# Autodesk Inventor assembly: chassis weldment bottom
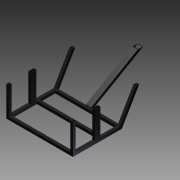
[picture p0: Inventor's stored thumbnail of the model, 180x180]
Saved by Autodesk Inventor 2012 (Build 160160000, 160)
## iProperties
Created: 2011-09-30
Part Number: chassis weldment bottom
Document SubType Name: Weldment
Designer: Antonella
Weld Material: Welded Aluminum-6061
Author: Antonella
## Documents named in this file (9)
- C:\Users\Antonella\Documents\GCC Robotics 2012 - Mechanical\Robot 2.0\Chassis\chassis weldment bottom.iam
- C:\Users\Antonella\Documents\GCC Robotics 2012 - Mechanical\Robot 2.0\Chassis\bottom frame member side.ipt
- C:\Users\Antonella\Documents\GCC Robotics 2012 - Mechanical\Robot 2.0\Chassis\bottom frame member crossbrace.ipt
- C:\Users\Antonella\Documents\GCC Robotics 2012 - Mechanical\Robot 2.0\Chassis\bottom frame member side_MIR.ipt
- C:\Users\Antonella\Documents\GCC Robotics 2012 - Mechanical\Robot 2.0\Chassis\bottom frame member angle.ipt
- C:\Users\Antonella\Documents\GCC Robotics 2012 - Mechanical\Robot 2.0\Chassis\bottom frame member back upright.ipt
- C:\Users\Antonella\Documents\GCC Robotics 2012 - Mechanical\Robot 2.0\Chassis\bottom frame member crossbrace back.ipt
- C:\Users\Antonella\Documents\GCC Robotics 2012 - Mechanical\Robot 2.0\Chassis\bottom frame member brace.ipt
- C:\Users\Antonella\Documents\GCC Robotics 2012 - Mechanical\Robot 2.0\Chassis\wheel mount vertical.ipt
## Components (12 placed, 8 different names)
1. bottom frame member side:1 — Mate:1, Flush:1, Mate:2, Mate:5, Flush:3, Mate:6, Flush:6, Flush:9, Mate:12, Flush:10, Mate:20, Flush:13
2. bottom frame member crossbrace:1 — Mate:1, Flush:1, Mate:2, Mate:3, Flush:2, Mate:4, Mate:9, Flush:5, Mate:10, Flush:7, Flush:17
3. bottom frame member side_MIR:1 — Mate:3, Flush:2, Mate:4, Mate:7, Flush:4, Mate:8, Flush:8, Mate:11, Mate:18, Flush:14
4. bottom frame member angle:1 — Mate:7, Flush:4, Mate:8
5. bottom frame member angle:2 — Mate:5, Flush:3, Mate:6
6. bottom frame member back upright:1 — Mate:10, Flush:7, Flush:8
7. bottom frame member back upright:2 — Mate:9, Flush:5, Flush:6
8. bottom frame member crossbrace back:1 — Mate:11, Flush:9, Mate:12, Mate:13, Mate:14, Mate:15, Mate:16, Mate:17
9. bottom frame member brace:1 — Mate:13, Mate:14, Mate:15
10. bottom frame member crossbrace back:2 — Mate:16, Flush:10, Mate:17
11. wheel mount vertical:1 — Mate:18, Flush:14, Flush:16, Flush:17
12. wheel mount vertical:2 — Mate:20, Flush:13, Flush:16
## Relationships (33: Mate 19, Flush 14)
- Mate:1: bottom frame member side:1 ↔ bottom frame member crossbrace:1
- Flush:1: bottom frame member side:1 ↔ bottom frame member crossbrace:1
- Mate:2: bottom frame member side:1 ↔ bottom frame member crossbrace:1
- Mate:3: bottom frame member crossbrace:1 ↔ bottom frame member side_MIR:1
- Flush:2: bottom frame member crossbrace:1 ↔ bottom frame member side_MIR:1
- Mate:4: bottom frame member crossbrace:1 ↔ bottom frame member side_MIR:1
- Mate:5: bottom frame member side:1 ↔ bottom frame member angle:2
- Flush:3: bottom frame member side:1 ↔ bottom frame member angle:2
- Mate:6: bottom frame member side:1 ↔ bottom frame member angle:2
- Mate:7: bottom frame member side_MIR:1 ↔ bottom frame member angle:1
- Flush:4: bottom frame member side_MIR:1 ↔ bottom frame member angle:1
- Mate:8: bottom frame member side_MIR:1 ↔ bottom frame member angle:1
- Mate:9: bottom frame member crossbrace:1 ↔ bottom frame member back upright:2
- Flush:5: bottom frame member crossbrace:1 ↔ bottom frame member back upright:2
- Flush:6: bottom frame member side:1 ↔ bottom frame member back upright:2
- Mate:10: bottom frame member crossbrace:1 ↔ bottom frame member back upright:1
- Flush:7: bottom frame member crossbrace:1 ↔ bottom frame member back upright:1
- Flush:8: bottom frame member side_MIR:1 ↔ bottom frame member back upright:1
- Mate:11: bottom frame member side_MIR:1 ↔ bottom frame member crossbrace back:1
- Flush:9: bottom frame member side:1 ↔ bottom frame member crossbrace back:1
- Mate:12: bottom frame member side:1 ↔ bottom frame member crossbrace back:1
- Mate:13: bottom frame member crossbrace back:1 ↔ bottom frame member brace:1
- Mate:14: bottom frame member crossbrace back:1 ↔ bottom frame member brace:1
- Mate:15: bottom frame member crossbrace back:1 ↔ bottom frame member brace:1
- Mate:16: bottom frame member crossbrace back:1 ↔ bottom frame member crossbrace back:2
- Flush:10: bottom frame member side:1 ↔ bottom frame member crossbrace back:2
- Mate:17 (-196.85 mm): bottom frame member crossbrace back:1 ↔ bottom frame member crossbrace back:2
- Mate:18: bottom frame member side_MIR:1 ↔ wheel mount vertical:1
- Mate:20: bottom frame member side:1 ↔ wheel mount vertical:2
- Flush:13: bottom frame member side:1 ↔ wheel mount vertical:2
- Flush:14: bottom frame member side_MIR:1 ↔ wheel mount vertical:1
- Flush:16: wheel mount vertical:1 ↔ wheel mount vertical:2
- Flush:17 (-231.14 mm): bottom frame member crossbrace:1 ↔ wheel mount vertical:1
